# Autodesk Inventor assembly: FinalExtruder
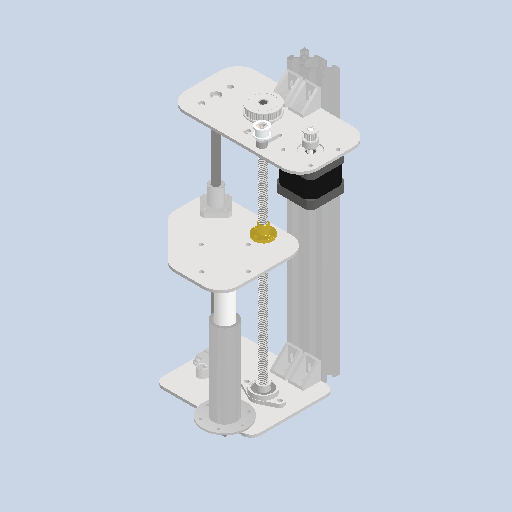
[picture p0: Inventor's stored thumbnail of the model, 512x512]
Saved by Autodesk Inventor 2025.2 (Build 292293000, 293)
## iProperties
Created: 2025-06-23
Part Number: FinalExtruder
Document SubType Name: Assembly
Designer: Simon
Author: Simon
## Documents named in this file (23)
- C:\Users\Simon\Projects\Hydrogel-3D-Printer\Hardware\Bioprinter Machine Design\Final System\Final Extruder\FinalExtruder.iam
- C:\Users\Simon\Projects\Hydrogel-3D-Printer\Hardware\Bioprinter Machine Design\PartsFolder\0.4 nozzle.ipt
- C:\Users\Simon\Projects\Hydrogel-3D-Printer\Hardware\Bioprinter Machine Design\PartsFolder\E3D-v6 Heater Block for Sensor Cartridges.ipt
- C:\Users\Simon\Projects\Hydrogel-3D-Printer\Hardware\Bioprinter Machine Design\Final System\Final Extruder\Plunger.ipt
- C:\Users\Simon\Projects\Hydrogel-3D-Printer\Hardware\Bioprinter Machine Design\Final System\Final Extruder\TR8x8-4_LeadScrew_285.ipt
- C:\Users\Simon\Projects\Hydrogel-3D-Printer\Hardware\Bioprinter Machine Design\PartsFolder\Stepper_17HS4401.ipt
- C:\Users\Simon\Projects\Hydrogel-3D-Printer\Hardware\Bioprinter Machine Design\PartsFolder\TR8x8-4_Nut.ipt
- C:\Users\Simon\Projects\Hydrogel-3D-Printer\Hardware\Bioprinter Machine Design\PartsFolder\GT2_16T_5.ipt
- C:\Users\Simon\Projects\Hydrogel-3D-Printer\Hardware\Bioprinter Machine Design\PartsFolder\GT2_48T_8.ipt
- C:\Users\Simon\Projects\Hydrogel-3D-Printer\Hardware\Bioprinter Machine Design\PartsFolder\Pillow Block Bearing 1\Zinc Alloy Pillow Block Flange Bearing KFL08 ID-8mm.iam
- C:\Users\Simon\Projects\Hydrogel-3D-Printer\Hardware\Bioprinter Machine Design\Final System\Final Extruder\2040_AluminimProfile_x.ipt
- C:\Users\Simon\Projects\Hydrogel-3D-Printer\Hardware\Bioprinter Machine Design\Final System\Final Extruder\CylinderAttachment.ipt
- C:\Users\Simon\Projects\Hydrogel-3D-Printer\Hardware\Bioprinter Machine Design\Final System\Final Extruder\SteelShaft_264.ipt
- C:\Users\Simon\Projects\Hydrogel-3D-Printer\Hardware\Bioprinter Machine Design\PartsFolder\SHF8.ipt
- C:\Users\Simon\Projects\Hydrogel-3D-Printer\Hardware\Bioprinter Machine Design\PartsFolder\LMK8UU.ipt
- C:\Users\Simon\Projects\Hydrogel-3D-Printer\Hardware\Bioprinter Machine Design\Final System\Final Extruder\TopMount.ipt
- C:\Users\Simon\Projects\Hydrogel-3D-Printer\Hardware\Bioprinter Machine Design\Final System\Final Extruder\MidMount.ipt
- C:\Users\Simon\Projects\Hydrogel-3D-Printer\Hardware\Bioprinter Machine Design\Final System\Final Extruder\BottomMount.ipt
- C:\Users\Simon\Projects\Hydrogel-3D-Printer\Hardware\Bioprinter Machine Design\PartsFolder\2020-corner-bracket.ipt
- C:\Users\Simon\Projects\Hydrogel-3D-Printer\Hardware\Bioprinter Machine Design\PartsFolder\Load Cell\50kg Load cell.iam
- C:\Users\Simon\Projects\Hydrogel-3D-Printer\Hardware\Bioprinter Machine Design\PartsFolder\GT2_20T_Smooth_Idler_5.ipt
- C:\Users\Simon\Projects\Hydrogel-3D-Printer\Hardware\Bioprinter Machine Design\PartsFolder\Spacer v2.ipt
- C:\Users\Simon\Projects\Hydrogel-3D-Printer\Hardware\Bioprinter Machine Design\Final System\Final Extruder\LoadCellMount.ipt
## Components (27 placed, 22 different names)
1. 0.4 nozzle:1 — Mate:1, Mate:2, Angle:1, Mate:19
2. E3D-v6 Heater Block for Sensor Cartridges:1 — Mate:1, Mate:2, Angle:1, Mate:18
3. TR8x8-4_LeadScrew_285:1 — Mate:7, Mate:9, Mate:11, Flush:1, Mate:22
4. Stepper_17HS4401:1 — Mate:10, Mate:29, Angle:2, Flush:8, Mate:52
5. TR8x8-4_Nut:2 — Mate:7, Mate:47, Mate:61, Mate:63
6. GT2_16T_5:1 — Mate:10, Flush:8, Flush:9
7. GT2_48T_8:1 — Mate:9, Flush:9, Flush:13
8. Zinc Alloy Pillow Block Flange Bearing KFL08 ID-8mm:1 [sub-assembly] — Mate:11, Flush:1, Mate:46, Angle:4
9. 2040_AluminimProfile_x:1 — Mate:14, Mate:15, Mate:16, Flush:5, Mate:25, Flush:7, Mate:27, Mate:33, Mate:35, Mate:41, Mate:43, Flush:10, Mate:49, Mate:50, Flush:11, Mate:51, Flush:12
10. Plunger:1 — Mate:65, Mate:69, Mate:72
11. CylinderAttachment:1 — Mate:18, Mate:19, Mate:32, Mate:57, Mate:58, Mate:65
12. Zinc Alloy Pillow Block Flange Bearing KFL08 ID-8mm:2 [sub-assembly] — Mate:22, Mate:31, Mate:53, Angle:3
13. SteelShaft_264:1 — Mate:23, Mate:24, Flush:3, Flush:4, Mate:45, Mate:54, Mate:60
14. SHF8:1 — Mate:23, Flush:3, Mate:56
15. SHF8:2 — Mate:24, Flush:4, Mate:30, Mate:55
16. LMK8UU:1 — Mate:45, Mate:48, Mate:62
17. TopMount:1 — Flush:5, Mate:25, Mate:29, Angle:2, Mate:30, Mate:31, Mate:34, Mate:36, Mate:52, Mate:53, Mate:54, Mate:55, Angle:3, Mate:64, Mate:66, Mate:67
18. MidMount:1 — Mate:47, Mate:48, Mate:60, Mate:61, Mate:62, Mate:63, Angle:5, Mate:70, Mate:71
19. BottomMount:1 — Flush:7, Mate:27, Mate:32, Mate:42, Mate:44, Mate:46, Flush:10, Mate:56, Angle:4, Mate:57, Mate:58
20. 2020-corner-bracket:1 — Mate:33, Mate:34, Mate:49
21. 2020-corner-bracket:2 — Mate:35, Mate:36, Mate:50, Flush:12
22. 2020-corner-bracket:5 — Mate:41, Mate:42, Mate:51
23. 2020-corner-bracket:6 — Mate:43, Mate:44, Flush:11
24. 50kg Load cell:1 [sub-assembly] — Mate:68, Angle:5, Mate:72
25. GT2_20T_Smooth_Idler_5:1 — Mate:64, Flush:13
26. Spacer v2:1 — Mate:66, Mate:67
27. LoadCellMount:1 — Mate:68, Mate:69, Mate:70, Mate:71
## Relationships (71: Mate 55, Flush 11, Angle 5)
- Mate:1: 0.4 nozzle:1 ↔ E3D-v6 Heater Block for Sensor Cartridges:1
- Mate:2: 0.4 nozzle:1 ↔ E3D-v6 Heater Block for Sensor Cartridges:1
- Angle:1 (0 deg): 0.4 nozzle:1 ↔ E3D-v6 Heater Block for Sensor Cartridges:1
- Mate:7: TR8x8-4_LeadScrew_285:1 ↔ TR8x8-4_Nut:2
- Mate:9: TR8x8-4_LeadScrew_285:1 ↔ GT2_48T_8:1
- Mate:10: Stepper_17HS4401:1 ↔ GT2_16T_5:1
- Mate:11: TR8x8-4_LeadScrew_285:1 ↔ Zinc Alloy Pillow Block Flange Bearing KFL08 ID-8mm:1
- Mate:14: 2040_AluminimProfile_x:1
- Mate:15: 2040_AluminimProfile_x:1
- Mate:16: 2040_AluminimProfile_x:1
- Mate:18: E3D-v6 Heater Block for Sensor Cartridges:1 ↔ CylinderAttachment:1
- Mate:19: 0.4 nozzle:1 ↔ CylinderAttachment:1
- Flush:1: TR8x8-4_LeadScrew_285:1 ↔ Zinc Alloy Pillow Block Flange Bearing KFL08 ID-8mm:1
- Mate:22: TR8x8-4_LeadScrew_285:1 ↔ Zinc Alloy Pillow Block Flange Bearing KFL08 ID-8mm:2
- Mate:23: SteelShaft_264:1 ↔ SHF8:1
- Mate:24: SteelShaft_264:1 ↔ SHF8:2
- Flush:3: SteelShaft_264:1 ↔ SHF8:1
- Flush:4: SteelShaft_264:1 ↔ SHF8:2
- Flush:5: 2040_AluminimProfile_x:1 ↔ TopMount:1
- Mate:25: 2040_AluminimProfile_x:1 ↔ TopMount:1
- Flush:7: 2040_AluminimProfile_x:1 ↔ BottomMount:1
- Mate:27: 2040_AluminimProfile_x:1 ↔ BottomMount:1
- Mate:29: Stepper_17HS4401:1 ↔ TopMount:1
- Angle:2 (90 deg): Stepper_17HS4401:1 ↔ TopMount:1
- Flush:8: Stepper_17HS4401:1 ↔ GT2_16T_5:1
- Mate:30: SHF8:2 ↔ TopMount:1
- Mate:31: Zinc Alloy Pillow Block Flange Bearing KFL08 ID-8mm:2 ↔ TopMount:1
- Mate:32: CylinderAttachment:1 ↔ BottomMount:1
- Flush:9: GT2_16T_5:1 ↔ GT2_48T_8:1
- Mate:33: 2040_AluminimProfile_x:1 ↔ 2020-corner-bracket:1
- Mate:34: TopMount:1 ↔ 2020-corner-bracket:1
- Mate:35: 2040_AluminimProfile_x:1 ↔ 2020-corner-bracket:2
- Mate:36: TopMount:1 ↔ 2020-corner-bracket:2
- Mate:41: 2040_AluminimProfile_x:1 ↔ 2020-corner-bracket:5
- Mate:42: BottomMount:1 ↔ 2020-corner-bracket:5
- Mate:43: 2040_AluminimProfile_x:1 ↔ 2020-corner-bracket:6
- Mate:44: BottomMount:1 ↔ 2020-corner-bracket:6
- Mate:45: SteelShaft_264:1 ↔ LMK8UU:1
- Mate:46: Zinc Alloy Pillow Block Flange Bearing KFL08 ID-8mm:1 ↔ BottomMount:1
- Flush:10: 2040_AluminimProfile_x:1 ↔ BottomMount:1
- Mate:47: TR8x8-4_Nut:2 ↔ MidMount:1
- Mate:48: LMK8UU:1 ↔ MidMount:1
- Mate:49: 2040_AluminimProfile_x:1 ↔ 2020-corner-bracket:1
- Mate:50: 2040_AluminimProfile_x:1 ↔ 2020-corner-bracket:2
- Flush:11: 2040_AluminimProfile_x:1 ↔ 2020-corner-bracket:6
- Mate:51: 2040_AluminimProfile_x:1 ↔ 2020-corner-bracket:5
- Flush:12 (-10 mm): 2040_AluminimProfile_x:1 ↔ 2020-corner-bracket:2
- Mate:52: Stepper_17HS4401:1 ↔ TopMount:1
- Mate:53: Zinc Alloy Pillow Block Flange Bearing KFL08 ID-8mm:2 ↔ TopMount:1
- Mate:54: SteelShaft_264:1 ↔ TopMount:1
- Mate:55: SHF8:2 ↔ TopMount:1
- Angle:3 (0 deg): Zinc Alloy Pillow Block Flange Bearing KFL08 ID-8mm:2 ↔ TopMount:1
- Mate:56: SHF8:1 ↔ BottomMount:1
- Angle:4 (0 deg): Zinc Alloy Pillow Block Flange Bearing KFL08 ID-8mm:1 ↔ BottomMount:1
- Mate:57: CylinderAttachment:1 ↔ BottomMount:1
- Mate:58: CylinderAttachment:1 ↔ BottomMount:1
- Mate:60: SteelShaft_264:1 ↔ MidMount:1
- Mate:61: TR8x8-4_Nut:2 ↔ MidMount:1
- Mate:62: LMK8UU:1 ↔ MidMount:1
- Mate:63: TR8x8-4_Nut:2 ↔ MidMount:1
- Mate:64: TopMount:1 ↔ GT2_20T_Smooth_Idler_5:1
- Flush:13: GT2_48T_8:1 ↔ GT2_20T_Smooth_Idler_5:1
- Mate:65: Plunger:1 ↔ CylinderAttachment:1
- Mate:66: TopMount:1 ↔ Spacer v2:1
- Mate:67: TopMount:1 ↔ Spacer v2:1
- Mate:68: 50kg Load cell:1 ↔ LoadCellMount:1
- Mate:69: Plunger:1 ↔ LoadCellMount:1
- Angle:5 (0 deg): MidMount:1 ↔ 50kg Load cell:1
- Mate:70: MidMount:1 ↔ LoadCellMount:1
- Mate:71: MidMount:1 ↔ LoadCellMount:1
- Mate:72: Plunger:1 ↔ 50kg Load cell:1
